# Autodesk Inventor assembly: PUll Tester with TFPX Plate
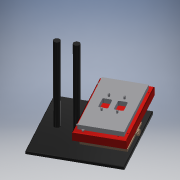
[picture p0: Inventor's stored thumbnail of the model, 180x180]
Saved by Autodesk Inventor 2019.4 (Build 234330000, 330)
## iProperties
Created: 2021-01-14
Part Number: PUll Tester with TFPX Plate
Document SubType Name: Assembly
Designer: caleb
Author: caleb
## Documents named in this file (3)
- C:\Users\cfang\Desktop\nebraska-silicon-lab\CAD\Pull Tester\PUll Tester with TFPX Plate.iam
- C:\Users\cfang\Desktop\nebraska-silicon-lab\CAD\TFPX\Wirebonding Plate\Plate Assembly.iam
- C:\Users\cfang\Desktop\nebraska-silicon-lab\CAD\Pull Tester\Pull Tester.iam
## Components (2 placed, 2 different names)
1. Plate Assembly:1 [sub-assembly] — Mate:1, Tangent:1, Tangent:2, Tangent:3
2. Pull Tester:1 [sub-assembly] — Mate:1, Tangent:1, Tangent:2, Tangent:3
## Relationships (4: Tangent 3, Mate 1)
- Mate:1: Plate Assembly:1 ↔ Pull Tester:1
- Tangent:1: Plate Assembly:1 ↔ Pull Tester:1
- Tangent:2: Plate Assembly:1 ↔ Pull Tester:1
- Tangent:3: Plate Assembly:1 ↔ Pull Tester:1
